# Autodesk Inventor assembly: ASY Beshkino_bio_tank
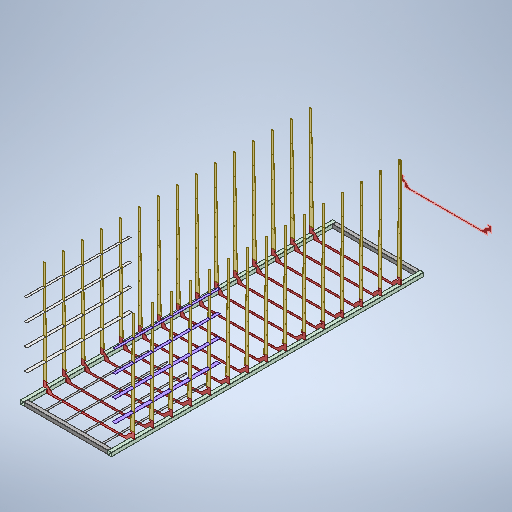
[picture p0: Inventor's stored thumbnail of the model, 512x512]
Saved by Autodesk Inventor 2025 (Build 290162010, 162A)
## iProperties
Created: 2024-07-21
Part Number: ASY Beshkino_bio_tank
Document SubType Name: Assembly
Designer: admin
Author: admin
## Documents named in this file (16)
- C:\Users\pokla\Documents\Inventor\BSH_Beshkino_bio_tank\ASY Beshkino_bio_tank.iam
- C:\Users\pokla\Documents\Inventor\BSH_Beshkino_bio_tank\BSH 000 dim Beshkino_bio_tank.ipt
- C:\Users\pokla\Documents\Inventor\BSH_Beshkino_bio_tank\BSH 010 floor 1.ipt
- C:\Users\pokla\Documents\Inventor\BSH_Beshkino_bio_tank\BSH 021 rib 1.ipt
- C:\Users\pokla\Documents\Inventor\BSH_Beshkino_bio_tank\BSH 022 rib 2.ipt
- C:\Users\pokla\Documents\Inventor\BSH_Beshkino_bio_tank\BSH 061 tube 1.ipt
- C:\Users\pokla\Documents\Inventor\BSH_Beshkino_bio_tank\BSH 031 nose 1.ipt
- C:\Users\pokla\Documents\Inventor\BSH_Beshkino_bio_tank\BSH 032 board 2.ipt
- C:\Users\pokla\Documents\Inventor\BSH_Beshkino_bio_tank\BSH 033 board 3.ipt
- C:\Users\pokla\Documents\Inventor\BSH_Beshkino_bio_tank\BSH 041 stringer 1.ipt
- C:\Users\pokla\Documents\Inventor\BSH_Beshkino_bio_tank\BSH 039 back 9.ipt
- C:\Users\pokla\Documents\Inventor\BSH_Beshkino_bio_tank\BSH 041 stringer floor.ipt
- C:\Users\pokla\Documents\Inventor\BSH_Beshkino_bio_tank\BSH 062 tube 2.ipt
- C:\Users\pokla\Documents\Inventor\BSH_Beshkino_bio_tank\BSH 042 stringer 2.ipt
- C:\Users\pokla\Documents\Inventor\BSH_Beshkino_bio_tank\BSH 043 stringer 3.ipt
- C:\Users\pokla\Documents\Inventor\BSH_Beshkino_bio_tank\BSH 044 stringer 4.ipt
## Components (73 placed, 15 different names)
1. BSH 000 dim Beshkino_bio_tank:1
2. BSH 010 floor 1:1 — Mate:5, Mate:6, Rigid:4, Mate:7, Flush:4, Mate:10, Flush:5
3. BSH 022 rib 2:1 — Rigid:3, Mate:8, Rigid:27, Rigid:28, Rigid:29, Rigid:30
4. BSH 061 tube 1:1 — Mate:1, Rigid:1, Mate:3, Flush:6
5. BSH 061 tube 1:2 — Mate:2, Rigid:1, Mate:4, Flush:3, Flush:4, Flush:14, Mate:14, Rigid:14, Rigid:15, Flush:15
6. BSH 031 nose 1:1 — Mate:10, Flush:5, Mate:11, Rigid:11
7. BSH 010 floor 1:2 — Rigid:4, Rigid:5
8. BSH 010 floor 1:3 — Rigid:5, Rigid:6, Mate:9
9. BSH 010 floor 1:4 — Rigid:6, Rigid:7
10. BSH 010 floor 1:5 — Rigid:7, Mate:12
11. BSH 032 board 2:1 — Mate:8, Mate:9, Rigid:8
12. BSH 033 board 3:1 — Rigid:8
13. BSH 031 nose 1:2 — Rigid:11
14. BSH 041 stringer 1:1 — Rigid:27
15. BSH 039 back 9:1 — Mate:12, Flush:6
16. BSH 020 rib 1:5 — Flush:14, Mate:14
17. BSH 041 stringer floor:1 — Rigid:20
18. BSH 062 tube 2:1 — Rigid:14
19. BSH 062 tube 2:2 — Rigid:15
20. BSH 022 rib 2:2 — Rigid:16, Rigid:31, Rigid:32, Rigid:33, Rigid:34
21. BSH 020 rib 1:1 — Mate:4, Flush:3, Mate:5, Mate:6, Rigid:3, Rigid:9, Flush:15, Rigid:16, Rigid:20, Rigid:22, Rigid:24, Rigid:26
22. BSH 041 stringer floor:3 — Rigid:22
23. BSH 041 stringer floor:5 — Rigid:24
24. BSH 041 stringer floor:7 — Rigid:26
25. BSH 042 stringer 2:1 — Rigid:28
26. BSH 043 stringer 3:1 — Rigid:29
27. BSH 044 stringer 4:1 — Rigid:30
28. BSH 041 stringer 1:2 — Rigid:31
29. BSH 042 stringer 2:2 — Rigid:32
30. BSH 043 stringer 3:2 — Rigid:33
31. BSH 044 stringer 4:2 — Rigid:34
32. BSH 022 rib 2:3 — Rigid:17
33. BSH 020 rib 1:3 — Rigid:9, Rigid:17, Rigid:18
34. BSH 022 rib 2:4 — Rigid:18
35. BSH 022 rib 2:5
36. BSH 020 rib 1:6
37. BSH 022 rib 2:6
38. BSH 022 rib 2:7
39. BSH 020 rib 1:7
40. BSH 022 rib 2:8
41. BSH 022 rib 2:9
42. BSH 020 rib 1:8
43. BSH 022 rib 2:10
44. BSH 022 rib 2:11
45. BSH 020 rib 1:9
46. BSH 022 rib 2:12
47. BSH 022 rib 2:13
48. BSH 020 rib 1:10
49. BSH 022 rib 2:14
50. BSH 022 rib 2:15
51. BSH 020 rib 1:11
52. BSH 022 rib 2:16
53. BSH 022 rib 2:17
54. BSH 020 rib 1:12
55. BSH 022 rib 2:18
56. BSH 022 rib 2:19
57. BSH 020 rib 1:13
58. BSH 022 rib 2:20
59. BSH 022 rib 2:21
60. BSH 020 rib 1:14
61. BSH 022 rib 2:22
62. BSH 022 rib 2:23
63. BSH 020 rib 1:15
64. BSH 022 rib 2:24
65. BSH 022 rib 2:25
66. BSH 020 rib 1:16
67. BSH 022 rib 2:26
68. BSH 022 rib 2:27
69. BSH 020 rib 1:17
70. BSH 022 rib 2:28
71. BSH 022 rib 2:29
72. BSH 020 rib 1:18
73. BSH 022 rib 2:30
## Component patterns: (14 elements, first: BSH 022 rib 2:3 + BSH 020 rib 1:3 + BSH 022 rib 2:4)
## Relationships (45: WeldJoint 26, Mate 13, Flush 6)
- Mate:1: BSH 061 tube 1:1
- Mate:2: BSH 061 tube 1:2
- Rigid:1 [WeldJoint] (-2400 mm): BSH 061 tube 1:1 ↔ BSH 061 tube 1:2
- Mate:3: BSH 061 tube 1:1
- Mate:4: BSH 061 tube 1:2 ↔ BSH 020 rib 1:1
- Flush:3: BSH 061 tube 1:2 ↔ BSH 020 rib 1:1
- Mate:5: BSH 010 floor 1:1 ↔ BSH 020 rib 1:1
- Mate:6: BSH 010 floor 1:1 ↔ BSH 020 rib 1:1
- Rigid:3 [WeldJoint]: BSH 022 rib 2:1 ↔ BSH 020 rib 1:1
- Rigid:4 [WeldJoint]: BSH 010 floor 1:1 ↔ BSH 010 floor 1:2
- Rigid:5 [WeldJoint]: BSH 010 floor 1:2 ↔ BSH 010 floor 1:3
- Rigid:6 [WeldJoint]: BSH 010 floor 1:3 ↔ BSH 010 floor 1:4
- Rigid:7 [WeldJoint]: BSH 010 floor 1:4 ↔ BSH 010 floor 1:5
- Mate:7: BSH 010 floor 1:1
- Flush:4 (100 mm): BSH 010 floor 1:1 ↔ BSH 061 tube 1:2
- Mate:8: BSH 022 rib 2:1 ↔ BSH 032 board 2:1
- Mate:9: BSH 010 floor 1:3 ↔ BSH 032 board 2:1
- Rigid:8 [WeldJoint]: BSH 032 board 2:1 ↔ BSH 033 board 3:1
- Rigid:9 [WeldJoint] (-500 mm): BSH 020 rib 1:1 ↔ BSH 020 rib 1:3
- Mate:10: BSH 010 floor 1:1 ↔ BSH 031 nose 1:1
- Flush:5 (10 mm): BSH 010 floor 1:1 ↔ BSH 031 nose 1:1
- Mate:11: BSH 031 nose 1:1
- Rigid:11 [WeldJoint]: BSH 031 nose 1:1 ↔ BSH 031 nose 1:2
- Mate:12: BSH 010 floor 1:5 ↔ BSH 039 back 9:1
- Flush:6: BSH 061 tube 1:1 ↔ BSH 039 back 9:1
- Flush:14: BSH 061 tube 1:2 ↔ BSH 020 rib 1:5
- Mate:14: BSH 061 tube 1:2 ↔ BSH 020 rib 1:5
- Rigid:14 [WeldJoint]: BSH 061 tube 1:2 ↔ BSH 062 tube 2:1
- Rigid:15 [WeldJoint]: BSH 061 tube 1:2 ↔ BSH 062 tube 2:2
- Flush:15 (598.5 mm): BSH 061 tube 1:2 ↔ BSH 020 rib 1:1
- Rigid:16 [WeldJoint]: BSH 022 rib 2:2 ↔ BSH 020 rib 1:1
- Rigid:17 [WeldJoint]: BSH 022 rib 2:3 ↔ BSH 020 rib 1:3
- Rigid:18 [WeldJoint]: BSH 020 rib 1:3 ↔ BSH 022 rib 2:4
- Rigid:20 [WeldJoint] (2 mm): BSH 041 stringer floor:1 ↔ BSH 020 rib 1:1
- Rigid:22 [WeldJoint] (2 mm): BSH 020 rib 1:1 ↔ BSH 041 stringer floor:3
- Rigid:24 [WeldJoint]: BSH 020 rib 1:1 ↔ BSH 041 stringer floor:5
- Rigid:26 [WeldJoint] (2 mm): BSH 020 rib 1:1 ↔ BSH 041 stringer floor:7
- Rigid:27 [WeldJoint] (2 mm): BSH 022 rib 2:1 ↔ BSH 041 stringer 1:1
- Rigid:28 [WeldJoint] (2 mm): BSH 022 rib 2:1 ↔ BSH 042 stringer 2:1
- Rigid:29 [WeldJoint] (2 mm): BSH 022 rib 2:1 ↔ BSH 043 stringer 3:1
- Rigid:30 [WeldJoint] (2 mm): BSH 022 rib 2:1 ↔ BSH 044 stringer 4:1
- Rigid:31 [WeldJoint] (2 mm): BSH 022 rib 2:2 ↔ BSH 041 stringer 1:2
- Rigid:32 [WeldJoint] (2 mm): BSH 022 rib 2:2 ↔ BSH 042 stringer 2:2
- Rigid:33 [WeldJoint] (2 mm): BSH 022 rib 2:2 ↔ BSH 043 stringer 3:2
- Rigid:34 [WeldJoint] (2 mm): BSH 022 rib 2:2 ↔ BSH 044 stringer 4:2
